# Autodesk Inventor assembly: flexMid
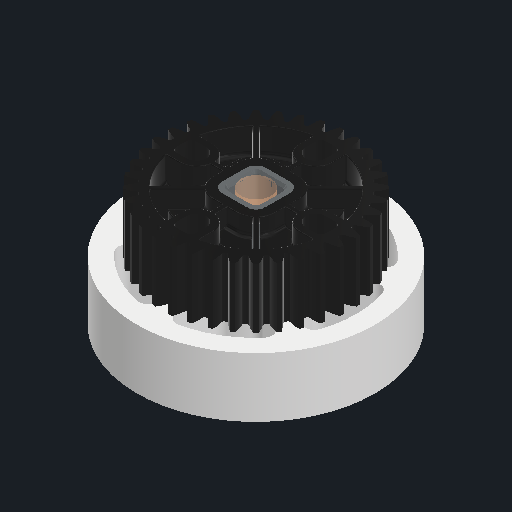
[picture p0: Inventor's stored thumbnail of the model, 512x512]
Saved by Autodesk Inventor 2024.2 (Build 282272000, 272)
## iProperties
Created: 2024-01-28
Part Number: flexMid
Document SubType Name: Assembly
Designer: reima
Author: reima
## Documents named in this file (5)
- O:\cad\61002g-cad\subasm\flexMid.iam
- O:\cad\61002g-cad\VEX parts\Motion\Wheels\Flex Wheels\2.000 Flex Wheel\2.000 30A .500.ipt
- O:\cad\61002g-cad\VEX parts\Motion\Wheels\Flex Wheels\2.000 Flex Wheel.ipt
- O:\cad\61002g-cad\VEX parts\Motion\Gears\HS Gear\HS 36T Gear, No Insert.iam
- O:\cad\61002g-cad\VEX parts\Motion\Gears\HS Gear.iam
## Components (2 placed, 2 different names)
1. 2.000 30A .500:1 — Insert:1
2. HS 36T Gear, No Insert:1 [sub-assembly] — Insert:1
## Relationships (1: Insert 1)
- Insert:1: 2.000 30A .500:1 ↔ HS 36T Gear, No Insert:1
